# Autodesk Inventor assembly: WheelAssembly
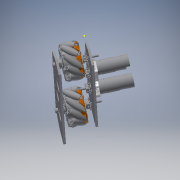
[picture p0: Inventor's stored thumbnail of the model, 180x180]
Saved by Autodesk Inventor 2017 (Build 210142000, 142)
## iProperties
Created: 2016-09-10
Part Number: WheelAssembly
Document SubType Name: Assembly
Designer: RoboticsUser
Author: RoboticsUser
## Documents named in this file (12)
- C:\Robotics\CAD\2016-17_CAD\WheelAssemble2.0 - left.iam
- C:\Robotics\CAD\COTSParts\Actobotics\545 parts\545556.ipt
- C:\Robotics\CAD\COTSParts\Actobotics\615 parts\615102.ipt
- C:\Robotics\CAD\COTSParts\Actobotics\634 parts\634080.ipt
- C:\Robotics\CAD\COTSParts\Motors\Andymark 2964  NeveRest 40 Motor.ipt
- C:\Robotics\CAD\COTSParts\Tetrix\tetrix-motor-mounts-1.snapshot.1\Tetrex 2pc motor mount.ipt
- C:\Robotics\CAD\COTSParts\Actobotics\545 parts\545456.ipt
- C:\Robotics\CAD\COTSParts\Wheels\AndyMark Mecanum Wheels\100mm Aluminum Mecanum wheels.ipt
- C:\Robotics\CAD\2016-17_CAD\DrainTrainPlate2.0.iam
- C:\Robotics\CAD\2016-17_CAD\DriveTrainPlate -Inside.ipt
- C:\Robotics\CAD\COTSParts\Actobotics\535 parts\535198.ipt
- C:\Robotics\CAD\COTSParts\Actobotics\collar.ipt
## Components (30 placed, 11 different names)
1. 545556:2 — Mate:10, Mate:13, Mate:47
2. 615102:4 — Insert:110
3. 634080:2 — Mate:10, Mate:12, Mate:26, Mate:45, Mate:56, Insert:103, Mate:65, Insert:117
4. 545556:6 — Insert:83, Mate:73
5. 634080:3 — Mate:28, Mate:50, Mate:66, Mate:68, Mate:71, Mate:74, Insert:118
6. Andymark 2964  NeveRest 40 Motor:2 — Insert:113, Mate:89
7. 545556:8 — Insert:112, Insert:113
8. 545556:9 — Insert:110, Insert:114
9. Andymark 2964  NeveRest 40 Motor:3 — Insert:111, Insert:114
10. Tetrex 2pc motor mount:1 — Mate:89, Mate:90, Mate:91
11. Tetrex 2pc motor mount:2 — Mate:80, Mate:81, Mate:82
12. 545456:1 — Mate:12, Mate:13, Insert:89
13. 545456:3 — Insert:83, Insert:88
14. 615102:6 — Insert:112
15. 615102:7 — Mate:45, Mate:47, Mate:70
16. 100mm Aluminum Mecanum wheels:1 — Insert:88, Mate:27, Mate:50
17. 100mm Aluminum Mecanum wheels:2 — Insert:89, Mate:25
18. 545456:4 — Mate:25, Mate:26, Insert:116
19. 545456:5 — Mate:27, Mate:28, Insert:115
20. 545556:12 — Insert:115, Mate:84
21. 545556:13 — Insert:116
22. DrainTrainPlate2.0:1 [sub-assembly] — Mate:56, Mate:65, Mate:66, Mate:68, Mate:84, Mate:85, Mate:86
23. DriveTrainPlate -Inside:1 — Insert:103, Mate:70, Mate:71, Insert:111, Mate:80, Mate:81, Mate:82, Mate:83, Mate:87, Mate:88, Mate:90, Mate:91
24. 615102:8 — Mate:73, Mate:74, Mate:83
25. 535198:2 — Mate:85
26. 535198:3 — Mate:88
27. 535198:4 — Mate:87
28. 535198:5 — Mate:86
29. collar:1 — Insert:117
30. collar:2 — Insert:118
## Relationships (43: Mate 30, Insert 13)
- Insert:83: 545556:6 ↔ 545456:3
- Mate:10: 545556:2 ↔ 634080:2
- Mate:12: 634080:2 ↔ 545456:1
- Mate:13: 545556:2 ↔ 545456:1
- Insert:88: 545456:3 ↔ 100mm Aluminum Mecanum wheels:1
- Insert:89: 545456:1 ↔ 100mm Aluminum Mecanum wheels:2
- Mate:25: 100mm Aluminum Mecanum wheels:2 ↔ 545456:4
- Mate:26: 634080:2 ↔ 545456:4
- Mate:27: 100mm Aluminum Mecanum wheels:1 ↔ 545456:5
- Mate:28: 634080:3 ↔ 545456:5
- Mate:45: 634080:2 ↔ 615102:7
- Mate:47: 545556:2 ↔ 615102:7
- Mate:50: 634080:3 ↔ 100mm Aluminum Mecanum wheels:1
- Mate:56: 634080:2 ↔ DrainTrainPlate2.0:1
- Insert:103 (36.0426 mm): 634080:2 ↔ DriveTrainPlate -Inside:1
- Mate:65 (-6.35 mm): 634080:2 ↔ DrainTrainPlate2.0:1
- Mate:66 (-6.35 mm): 634080:3 ↔ DrainTrainPlate2.0:1
- Mate:68: 634080:3 ↔ DrainTrainPlate2.0:1
- Mate:70 (3.175 mm): 615102:7 ↔ DriveTrainPlate -Inside:1
- Mate:71 (6.35 mm): 634080:3 ↔ DriveTrainPlate -Inside:1
- Mate:73: 545556:6 ↔ 615102:8
- Mate:74: 634080:3 ↔ 615102:8
- Insert:110: 615102:4 ↔ 545556:9
- Insert:111 (25.4 mm): Andymark 2964  NeveRest 40 Motor:3 ↔ DriveTrainPlate -Inside:1
- Insert:114 (2.4638 mm): 545556:9 ↔ Andymark 2964  NeveRest 40 Motor:3
- Mate:80: Tetrex 2pc motor mount:2 ↔ DriveTrainPlate -Inside:1
- Mate:81: Tetrex 2pc motor mount:2 ↔ DriveTrainPlate -Inside:1
- Mate:82: Tetrex 2pc motor mount:2 ↔ DriveTrainPlate -Inside:1
- Insert:112 (-2.6416 mm): 545556:8 ↔ 615102:6
- Insert:113: Andymark 2964  NeveRest 40 Motor:2 ↔ 545556:8
- Insert:115: 545456:5 ↔ 545556:12
- Mate:83 (3.175 mm): DriveTrainPlate -Inside:1 ↔ 615102:8
- Mate:84: 545556:12 ↔ DrainTrainPlate2.0:1
- Insert:116: 545456:4 ↔ 545556:13
- Mate:85: DrainTrainPlate2.0:1 ↔ 535198:2
- Mate:86: DrainTrainPlate2.0:1 ↔ 535198:5
- Mate:87: DriveTrainPlate -Inside:1 ↔ 535198:4
- Mate:88: DriveTrainPlate -Inside:1 ↔ 535198:3
- Insert:117: 634080:2 ↔ collar:1
- Insert:118 (-6.35 mm): 634080:3 ↔ collar:2
- Mate:89: Andymark 2964  NeveRest 40 Motor:2 ↔ Tetrex 2pc motor mount:1
- Mate:90: Tetrex 2pc motor mount:1 ↔ DriveTrainPlate -Inside:1
- Mate:91: Tetrex 2pc motor mount:1 ↔ DriveTrainPlate -Inside:1
